# Autodesk Inventor assembly: Overview
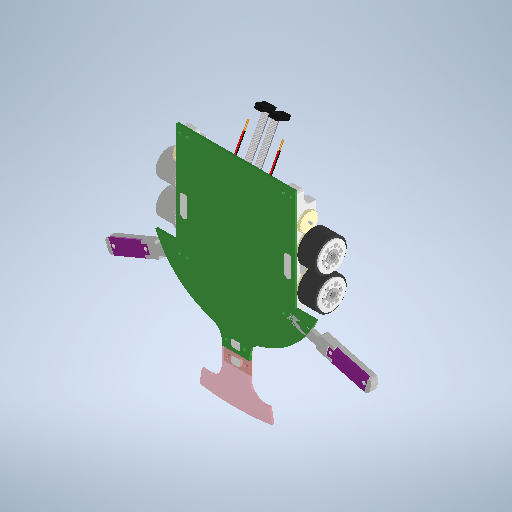
[picture p0: Inventor's stored thumbnail of the model, 512x512]
Saved by Autodesk Inventor 2025 (Build 290162000, 162)
## iProperties
Created: 2021-10-05
Part Number: Overview
Document SubType Name: Assembly
Designer: shiok
Mass: 68.0359 g
Surface Area: 547.496 cm^2
Volume: 44.6592 cm^3
Author: shiok
## Documents named in this file (11)
- C:\Users\yazawa\Documents\git\murakumo\inventor\Overview.iam
- C:\Users\yazawa\Documents\git\murakumo\inventor\flame.ipt
- C:\Users\yazawa\Documents\git\murakumo\inventor\sensor.ipt
- C:\Users\yazawa\Documents\git\murakumo\inventor\SideSensorCircuit.ipt
- C:\Users\yazawa\Documents\git\murakumo\inventor\top.ipt
- C:\Users\yazawa\Documents\git\murakumo\inventor\jump.ipt
- C:\Users\yazawa\Documents\git\murakumo\inventor\SideSensor_Mount.ipt
- C:\Users\yazawa\Documents\git\murakumo\inventor\Motor.iam
- C:\Users\yazawa\Documents\git\murakumo\inventor\battery.ipt
- C:\Users\yazawa\Documents\git\murakumo\inventor\SideSensorCircuit_MIR4.ipt
- C:\Users\yazawa\Documents\git\murakumo\inventor\Motor_MIR.iam
## Components (11 placed, 10 different names)
1. flame:1 — フラッシュ:1, フラッシュ:2, フラッシュ:3, メイト:15, フラッシュ:7, メイト:16, メイト:23, メイト:24, メイト:25, メイト:30, メイト:31, メイト:34, メイト:35, メイト:36
2. sensor:1 — フラッシュ:6, メイト:15, フラッシュ:7, メイト:17, メイト:18
3. top:1 — メイト:26, メイト:27, メイト:28
4. jump:1 — メイト:16, メイト:17, メイト:18
5. SideSensorCircuit:1 — メイト:19, フラッシュ:8, 挿入:22, メイト:37, メイト:38, メイト:39
6. SideSensor_Mount:1 — メイト:19, フラッシュ:8, 挿入:22, メイト:29, メイト:30, メイト:35, メイト:36, メイト:37, メイト:38, メイト:39
7. Motor:1 [sub-assembly] — メイト:23, メイト:24, メイト:25, メイト:26, メイト:27, メイト:28, メイト:29
8. battery:1 — メイト:31, フラッシュ:9
9. SideSensorCircuit_MIR4:1 — 挿入:24, 挿入:25, フラッシュ:10, メイト:32
10. SideSensor_Mount:2 — 挿入:24, 挿入:25, フラッシュ:10, メイト:32, メイト:33, メイト:34
11. Motor_MIR:1 [sub-assembly] — メイト:33
## Relationships (33: Mate 22, Flush 8, Insert 3)
- フラッシュ:1 [Flush]: flame:1
- フラッシュ:2 [Flush]: flame:1
- フラッシュ:3 [Flush]: flame:1
- フラッシュ:6 [Flush]: sensor:1
- メイト:15 [Mate]: flame:1 ↔ sensor:1
- フラッシュ:7 [Flush]: flame:1 ↔ sensor:1
- メイト:16 [Mate]: flame:1 ↔ jump:1
- メイト:17 [Mate]: sensor:1 ↔ jump:1
- メイト:18 [Mate]: sensor:1 ↔ jump:1
- メイト:19 [Mate]: SideSensorCircuit:1 ↔ SideSensor_Mount:1
- フラッシュ:8 [Flush]: SideSensorCircuit:1 ↔ SideSensor_Mount:1
- 挿入:22 [Insert]: SideSensorCircuit:1 ↔ SideSensor_Mount:1
- メイト:23 [Mate]: flame:1 ↔ Motor:1
- メイト:24 [Mate]: flame:1 ↔ Motor:1
- メイト:25 [Mate]: flame:1 ↔ Motor:1
- メイト:26 [Mate]: top:1 ↔ Motor:1
- メイト:27 [Mate]: top:1 ↔ Motor:1
- メイト:28 [Mate]: top:1 ↔ Motor:1
- メイト:29 [Mate]: SideSensor_Mount:1 ↔ Motor:1
- メイト:30 [Mate]: flame:1 ↔ SideSensor_Mount:1
- メイト:31 [Mate]: flame:1 ↔ battery:1
- フラッシュ:9 [Flush]: battery:1
- 挿入:24 [Insert]: SideSensorCircuit_MIR4:1 ↔ SideSensor_Mount:2
- 挿入:25 [Insert]: SideSensorCircuit_MIR4:1 ↔ SideSensor_Mount:2
- フラッシュ:10 [Flush]: SideSensorCircuit_MIR4:1 ↔ SideSensor_Mount:2
- メイト:32 [Mate]: SideSensorCircuit_MIR4:1 ↔ SideSensor_Mount:2
- メイト:33 [Mate]: SideSensor_Mount:2 ↔ Motor_MIR:1
- メイト:34 [Mate]: flame:1 ↔ SideSensor_Mount:2
- メイト:35 [Mate]: flame:1 ↔ SideSensor_Mount:1
- メイト:36 [Mate]: flame:1 ↔ SideSensor_Mount:1
- メイト:37 [Mate]: SideSensorCircuit:1 ↔ SideSensor_Mount:1
- メイト:38 [Mate]: SideSensorCircuit:1 ↔ SideSensor_Mount:1
- メイト:39 [Mate]: SideSensorCircuit:1 ↔ SideSensor_Mount:1
